# Autodesk Inventor assembly: a_frame_oko
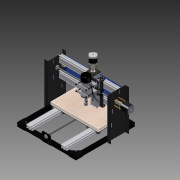
[picture p0: Inventor's stored thumbnail of the model, 180x180]
Saved by Autodesk Inventor 2014 (Build 180170000, 170)
## iProperties
Created: 2013-07-14
Part Number: a_frame_oko
Document SubType Name: Assembly
Designer: Edward
Mass: 4088.46 g
Surface Area: 15664.1 cm^2
Volume: 2491 cm^3
Density: 1.64129 g/cm^3
Author: Edward
## Documents named in this file (29)
- C:\Users\Edward\Desktop\Shapeoko_2.0_collection\Shapeoko_bm\a_frame_oko.iam
- C:\Users\Edward\Desktop\Shapeoko_2.0_collection\Shapeoko_bm\S2_MS400.ipt
- C:\Users\Edward\Desktop\Shapeoko_2.0_collection\Shapeoko_bm\hfs5_2020_400.ipt
- C:\Users\Edward\Desktop\Shapeoko_2.0_collection\Shapeoko_bm\x-carriage.ipt
- C:\Users\Edward\Desktop\Shapeoko_2.0_collection\Shapeoko_bm\y-carriage.ipt
- C:\Users\Edward\Desktop\Shapeoko_2.0_collection\Shapeoko_bm\hfs5_2020_360.ipt
- C:\Users\Edward\Desktop\Shapeoko_2.0_collection\Shapeoko_bm\SM-E01.ipt
- C:\Users\Edward\Desktop\Shapeoko_2.0_collection\Shapeoko_bm\SM-M08.ipt
- C:\Users\Edward\Desktop\Shapeoko_2.0_collection\Shapeoko_bm\B30037.iam
- C:\Users\Edward\Desktop\Shapeoko_2.0_collection\Shapeoko_bm\SM-H10.ipt
- C:\Users\Edward\Desktop\Shapeoko_2.0_collection\Shapeoko_bm\SM-H12.ipt
- C:\Users\Edward\Desktop\Shapeoko_2.0_collection\Shapeoko_bm\wasteboard.ipt
- C:\Users\Edward\Desktop\Shapeoko_2.0_collection\Shapeoko_bm\B18033.ipt
- C:\Users\Edward\Desktop\Shapeoko_2.0_collection\Shapeoko_bm\frame_gusset.ipt
- C:\Users\Edward\Desktop\Shapeoko_2.0_collection\Shapeoko_bm\93655A021.ipt
- C:\Users\Edward\Desktop\Shapeoko_2.0_collection\Shapeoko_bm\hblsd_assembly.iam
- C:\Users\Edward\Desktop\Shapeoko_2.0_collection\Shapeoko_bm\7804K145.ipt
- C:\Users\Edward\Desktop\Shapeoko_2.0_collection\Shapeoko_bm\part_plate_rear.ipt
- C:\Users\Edward\Desktop\Shapeoko_2.0_collection\Shapeoko_bm\91239A233.ipt
- C:\Users\Edward\Desktop\Shapeoko_2.0_collection\Shapeoko_bm\SM-H03.ipt
- C:\Users\Edward\Desktop\Shapeoko_2.0_collection\Shapeoko_bm\revamped_simple_z-axis_assembly.iam
- C:\Users\Edward\Desktop\Shapeoko_2.0_collection\Shapeoko_bm\simple_upright.ipt
- C:\Users\Edward\Desktop\Shapeoko_2.0_collection\Shapeoko_bm\z-bearing.ipt
- C:\Users\Edward\Desktop\Shapeoko_2.0_collection\Shapeoko_bm\nema17_y_axis_motor_mount_12ga.ipt
- C:\Users\Edward\Desktop\Shapeoko_2.0_collection\Shapeoko_bm\Imported Components\iec320_703W-00_04\iec320_703W-00_04.ipt
- C:\Users\Edward\Desktop\Shapeoko_2.0_collection\Shapeoko_bm\Imported Components\Arduino\Arduino.ipt
- C:\Users\Edward\Desktop\Shapeoko_2.0_collection\Shapeoko_bm\x_acme_upgrade.ipt
- C:\Users\Edward\Desktop\Shapeoko_2.0_collection\Shapeoko_bm\Imported Components\92844-005 USB CABLE B MALE TO B FEMALE PANEL MOUNT\92844-005 USB CABLE B MALE TO B FEMALE PANEL MOUNT.ipt
- C:\Users\Edward\Desktop\Shapeoko_2.0_collection\Shapeoko_bm\23015T81_leveling_feet.ipt
## Components (93 placed, 28 different names)
1. S2_MS400:1 — Mate:2, Flush:2, Flush:5, Mate:61, Flush:49, Mate:65, Flush:51
2. S2_MS400:2 — Mate:1, Flush:1, Mate:3, Flush:4, Mate:15, Mate:63, Flush:50, Mate:67, Flush:52
3. S2_MS400:3 — Flush:13, Flush:14, Flush:16, Angle:5, Insert:68, Insert:70
4. S2_MS400:4 — Flush:13, Flush:14, Mate:81, Flush:64, Mate:86, Flush:66, Insert:67, Flush:70, Insert:69, Mate:93, Flush:73
5. hfs5_2020_360:1 — Mate:1, Mate:2, Flush:1, Flush:2, Flush:3, Mate:4, Mate:5, Flush:6, Flush:7, Flush:8, Flush:9, Mate:39, Flush:33, Flush:37, Flush:40, Mate:64, Mate:66, Mate:95, Flush:74
6. hfs5_2020_360:2 — Mate:3, Flush:3, Flush:4, Flush:5, Flush:16, Mate:26, Flush:25, Flush:42, Flush:44, Flush:45, Flush:48, Mate:60, Mate:62
7. hfs5_2020_400:3 — Mate:4, Flush:8, Flush:9, Flush:34, Mate:45, Mate:54, Mate:55, Flush:46, Flush:47, Mate:90, Flush:71, Flush:77
8. hfs5_2020_400:4 — Mate:5, Flush:6, Flush:7, Flush:26, Mate:50, Mate:51, Flush:38, Flush:39, Mate:52, Flush:41, Mate:53, Flush:43, Mate:91, Flush:72
9. y-carriage:1 — Mate:15, Mate:20, Flush:20, Flush:21, Mate:36, Flush:31, Flush:32, Insert:3, Insert:4, Insert:5, Insert:6, Insert:7, Insert:8, Insert:9, Insert:10, Mate:41, Mate:44, Mate:57, Mate:59
10. SM-E01:2 — Mate:23, Insert:30, Insert:31, Insert:32, Insert:33, Mate:92, Mate:105
11. SM-M08:1 — Mate:20, Flush:20, Flush:21, Mate:28
12. SM-M08:2 — Mate:23, Flush:63, Mate:102
13. nema17_y_axis_motor_mount_12ga:1 — Mate:26, Flush:25, Flush:26, Angle:2, Mate:46, Angle:3, Angle:5, Insert:76, Flush:78
14. SM-E01:3 — Mate:28, Angle:2, Mate:30, Mate:46, Angle:3, Insert:20, Insert:21, Insert:24, Insert:25
15. SM-H12:1 — Mate:30, Mate:101
16. x_acme_upgrade:2 — Insert:81, Mate:101
17. x_acme_upgrade:1 — Mate:102, Insert:82
18. wasteboard:1 — Mate:36, Flush:31, Flush:32
19. B30037:5 [sub-assembly] — Insert:3
20. B30037:6 [sub-assembly] — Insert:4, Insert:64
21. B30037:7 [sub-assembly] — Insert:5, Insert:66
22. B30037:8 [sub-assembly] — Insert:6
23. B18033:1 — Insert:7, Mate:58
24. B18033:2 — Insert:8, Mate:56
25. B18033:3 — Insert:9, Mate:43
26. B18033:4 — Insert:10, Mate:40
27. B30037:9 [sub-assembly] — Mate:58, Mate:59, Insert:63
28. B30037:10 [sub-assembly] — Mate:40, Mate:41
29. B30037:11 [sub-assembly] — Mate:43, Mate:44
30. B30037:12 [sub-assembly] — Mate:56, Mate:57, Insert:65
31. frame_gusset:1 — Mate:39, Flush:33, Flush:34, Flush:35, Flush:36
32. frame_gusset:2 — Mate:45, Flush:35, Flush:36, Insert:83
33. frame_gusset:3 — Mate:51, Flush:37, Flush:38
34. frame_gusset:4 — Mate:50, Flush:39, Flush:40, Insert:84
35. frame_gusset:5 — Mate:52, Flush:41, Flush:42
36. frame_gusset:6 — Mate:53, Flush:43, Flush:44, Insert:85
37. frame_gusset:7 — Mate:55, Flush:45, Flush:46, Insert:86
38. frame_gusset:8 — Mate:54, Flush:47, Flush:48
39. 93655A021:1 — Insert:22
40. 93655A021:2 — Insert:19, Insert:21
41. 93655A021:3 — Insert:19
42. 93655A021:4 — Insert:18, Insert:20
43. 93655A021:5 — Insert:18
44. 93655A021:6 — Insert:22, Insert:25
45. 93655A021:7 — Insert:23
46. 93655A021:8 — Insert:23, Insert:24
47. hblsd_assembly:1 [sub-assembly] — Mate:64, Mate:65, Flush:51
48. hblsd_assembly:2 [sub-assembly] — Mate:66, Mate:67, Flush:52
49. hblsd_assembly:3 [sub-assembly] — Mate:62, Mate:63, Flush:50
50. hblsd_assembly:4 [sub-assembly] — Mate:60, Mate:61, Flush:49
51. 93655A021:9 — Insert:31
52. 93655A021:10
53. 93655A021:11 — Insert:33
54. 93655A021:12
55. 93655A021:13 — Insert:32
56. 93655A021:14
57. 93655A021:15 — Insert:30
58. 93655A021:16 — Insert:75
59. 7804K145:1 — Insert:55
60. B30037:14 [sub-assembly] — Insert:51
61. B30037:15 [sub-assembly] — Insert:52
62. x-carriage:2 — Mate:81, Flush:63, Flush:64, Insert:51, Insert:52, Insert:53, Insert:54, Mate:83, Mate:85, Mate:89, Flush:68, Flush:69
63. B18033:5 — Insert:53, Mate:84
64. B18033:6 — Insert:54, Mate:82
65. B30037:16 [sub-assembly] — Mate:82, Mate:83
66. B30037:17 [sub-assembly] — Mate:84, Mate:85
67. SM-H10:12 — Insert:55
68. part_plate_rear:1 — Mate:86, Flush:66
69. 91239A233:1 — Insert:59
70. SM-H03:1 — Insert:59, Insert:65
71. 91239A233:2
72. SM-H03:2 — Insert:63
73. 91239A233:3
74. SM-H03:3 — Insert:66
75. 91239A233:4
76. SM-H03:4 — Insert:64
77. revamped_simple_z-axis_assembly:1 [sub-assembly] — Mate:89, Flush:68, Flush:69
78. simple_upright:1 — Mate:90, Insert:67, Flush:70, Flush:71, Insert:68, Insert:71, Insert:75, Flush:77
79. simple_upright:2 — Mate:91, Flush:72, Insert:69, Insert:70, Insert:72, Mate:97, Flush:76, Mate:98, Mate:103
80. z-bearing:1 — Insert:71
81. z-bearing:2 — Insert:72, Mate:92, Insert:82
82. part_plate_rear:2 — Mate:93, Flush:73, Mate:100, Flush:79
83. z-bearing:3 — Insert:76
84. nema17_y_axis_motor_mount_12ga:2 — Insert:78, Mate:95, Flush:74, Flush:78
85. z-bearing:4 — Insert:78, Insert:81
86. SM-H12:3 — Mate:105
87. iec320_703W-00_04:1 — Mate:97, Flush:76, Mate:98
88. Arduino:1 — Mate:100, Flush:79
89. 92844-005 USB CABLE B MALE TO B FEMALE PANEL MOUNT:1 — Mate:103
90. 23015T81_leveling_feet:1 — Insert:83
91. 23015T81_leveling_feet:2 — Insert:84
92. 23015T81_leveling_feet:3 — Insert:85
93. 23015T81_leveling_feet:4 — Insert:86
## Relationships (163: Mate 56, Flush 52, Insert 52, Angle 3)
- Mate:1: S2_MS400:2 ↔ hfs5_2020_360:1
- Mate:2: S2_MS400:1 ↔ hfs5_2020_360:1
- Flush:1: S2_MS400:2 ↔ hfs5_2020_360:1
- Flush:2: S2_MS400:1 ↔ hfs5_2020_360:1
- Mate:3: S2_MS400:2 ↔ hfs5_2020_360:2
- Flush:3: hfs5_2020_360:1 ↔ hfs5_2020_360:2
- Flush:4: S2_MS400:2 ↔ hfs5_2020_360:2
- Flush:5: S2_MS400:1 ↔ hfs5_2020_360:2
- Mate:4: hfs5_2020_360:1 ↔ hfs5_2020_400:3
- Mate:5: hfs5_2020_360:1 ↔ hfs5_2020_400:4
- Flush:6: hfs5_2020_360:1 ↔ hfs5_2020_400:4
- Flush:7: hfs5_2020_360:1 ↔ hfs5_2020_400:4
- Flush:8: hfs5_2020_360:1 ↔ hfs5_2020_400:3
- Flush:9: hfs5_2020_360:1 ↔ hfs5_2020_400:3
- Flush:13: S2_MS400:3 ↔ S2_MS400:4
- Flush:14 (90 mm): S2_MS400:3 ↔ S2_MS400:4
- Mate:15 (6.35 mm): S2_MS400:2 ↔ y-carriage:1
- Flush:16 (95.5 mm): S2_MS400:3 ↔ hfs5_2020_360:2
- Mate:20: y-carriage:1 ↔ SM-M08:1
- Flush:20 (90 mm): y-carriage:1 ↔ SM-M08:1
- Flush:21 (142.5 mm): y-carriage:1 ↔ SM-M08:1
- Mate:23: SM-E01:2 ↔ SM-M08:2
- Mate:26: hfs5_2020_360:2 ↔ nema17_y_axis_motor_mount_12ga:1
- Flush:25: hfs5_2020_360:2 ↔ nema17_y_axis_motor_mount_12ga:1
- Flush:26 (170 mm): hfs5_2020_400:4 ↔ nema17_y_axis_motor_mount_12ga:1
- Mate:28: SM-M08:1 ↔ SM-E01:3
- Angle:2 (0 deg): nema17_y_axis_motor_mount_12ga:1 ↔ SM-E01:3
- Mate:30: SM-E01:3 ↔ SM-H12:1
- Mate:36: y-carriage:1 ↔ wasteboard:1
- Flush:31: y-carriage:1 ↔ wasteboard:1
- Flush:32: y-carriage:1 ↔ wasteboard:1
- Insert:3 (1 mm): y-carriage:1 ↔ B30037:5
- Insert:4 (1 mm): y-carriage:1 ↔ B30037:6
- Insert:5 (1 mm): y-carriage:1 ↔ B30037:7
- Insert:6 (1 mm): y-carriage:1 ↔ B30037:8
- Insert:7: y-carriage:1 ↔ B18033:1
- Insert:8: y-carriage:1 ↔ B18033:2
- Insert:9: y-carriage:1 ↔ B18033:3
- Insert:10: y-carriage:1 ↔ B18033:4
- Mate:39: hfs5_2020_360:1 ↔ frame_gusset:1
- Flush:33: hfs5_2020_360:1 ↔ frame_gusset:1
- Flush:34: hfs5_2020_400:3 ↔ frame_gusset:1
- Mate:40: B18033:4 ↔ B30037:10
- Mate:41 (1 mm): y-carriage:1 ↔ B30037:10
- Mate:43: B18033:3 ↔ B30037:11
- Mate:44 (1 mm): y-carriage:1 ↔ B30037:11
- Mate:45: hfs5_2020_400:3 ↔ frame_gusset:2
- Flush:35: frame_gusset:1 ↔ frame_gusset:2
- Flush:36: frame_gusset:1 ↔ frame_gusset:2
- Mate:46 (50 mm): nema17_y_axis_motor_mount_12ga:1 ↔ SM-E01:3
- Angle:3 (0 deg): nema17_y_axis_motor_mount_12ga:1 ↔ SM-E01:3
- Mate:50: hfs5_2020_400:4 ↔ frame_gusset:4
- Mate:51: hfs5_2020_400:4 ↔ frame_gusset:3
- Flush:37: hfs5_2020_360:1 ↔ frame_gusset:3
- Flush:38: hfs5_2020_400:4 ↔ frame_gusset:3
- Flush:39: hfs5_2020_400:4 ↔ frame_gusset:4
- Flush:40: hfs5_2020_360:1 ↔ frame_gusset:4
- Mate:52: hfs5_2020_400:4 ↔ frame_gusset:5
- Flush:41: hfs5_2020_400:4 ↔ frame_gusset:5
- Flush:42: hfs5_2020_360:2 ↔ frame_gusset:5
- Mate:53: hfs5_2020_400:4 ↔ frame_gusset:6
- Flush:43: hfs5_2020_400:4 ↔ frame_gusset:6
- Flush:44: hfs5_2020_360:2 ↔ frame_gusset:6
- Mate:54: hfs5_2020_400:3 ↔ frame_gusset:8
- Mate:55: hfs5_2020_400:3 ↔ frame_gusset:7
- Flush:45: hfs5_2020_360:2 ↔ frame_gusset:7
- Flush:46: hfs5_2020_400:3 ↔ frame_gusset:7
- Flush:47: hfs5_2020_400:3 ↔ frame_gusset:8
- Flush:48: hfs5_2020_360:2 ↔ frame_gusset:8
- Mate:56: B18033:2 ↔ B30037:12
- Mate:57 (1 mm): y-carriage:1 ↔ B30037:12
- Mate:58: B18033:1 ↔ B30037:9
- Mate:59 (1 mm): y-carriage:1 ↔ B30037:9
- Insert:18: 93655A021:4 ↔ 93655A021:5
- Insert:19: 93655A021:2 ↔ 93655A021:3
- Insert:20: SM-E01:3 ↔ 93655A021:4
- Insert:21: SM-E01:3 ↔ 93655A021:2
- Insert:22: 93655A021:1 ↔ 93655A021:6
- Insert:23: 93655A021:7 ↔ 93655A021:8
- Insert:24: SM-E01:3 ↔ 93655A021:8
- Insert:25: SM-E01:3 ↔ 93655A021:6
- Mate:60: hfs5_2020_360:2 ↔ hblsd_assembly:4
- Mate:61: S2_MS400:1 ↔ hblsd_assembly:4
- Flush:49 (3 mm): S2_MS400:1 ↔ hblsd_assembly:4
- Mate:62: hfs5_2020_360:2 ↔ hblsd_assembly:3
- Mate:63: S2_MS400:2 ↔ hblsd_assembly:3
- Flush:50 (3 mm): S2_MS400:2 ↔ hblsd_assembly:3
- Mate:64: hfs5_2020_360:1 ↔ hblsd_assembly:1
- Mate:65: S2_MS400:1 ↔ hblsd_assembly:1
- Flush:51 (3 mm): S2_MS400:1 ↔ hblsd_assembly:1
- Mate:66: hfs5_2020_360:1 ↔ hblsd_assembly:2
- Mate:67: S2_MS400:2 ↔ hblsd_assembly:2
- Flush:52 (3 mm): S2_MS400:2 ↔ hblsd_assembly:2
- [Insert]: 93655A021:9 ↔ 93655A021:10
- [Insert]: 93655A021:11 ↔ 93655A021:12
- [Insert]: 93655A021:13 ↔ 93655A021:14
- [Insert]: 93655A021:15 ↔ 93655A021:16
- Insert:30: SM-E01:2 ↔ 93655A021:15
- Insert:31: SM-E01:2 ↔ 93655A021:9
- Insert:32: SM-E01:2 ↔ 93655A021:13
- Insert:33: SM-E01:2 ↔ 93655A021:11
- Angle:5 (0 deg): S2_MS400:3 ↔ nema17_y_axis_motor_mount_12ga:1
- Mate:81 (6.35 mm): S2_MS400:4 ↔ x-carriage:2
- Flush:63: SM-M08:2 ↔ x-carriage:2
- Flush:64 (-22.5 mm): S2_MS400:4 ↔ x-carriage:2
- Insert:51 (1 mm): B30037:14 ↔ x-carriage:2
- Insert:52 (1 mm): B30037:15 ↔ x-carriage:2
- Insert:53: x-carriage:2 ↔ B18033:5
- Insert:54: x-carriage:2 ↔ B18033:6
- Mate:82: B18033:6 ↔ B30037:16
- Mate:83 (1 mm): x-carriage:2 ↔ B30037:16
- Mate:84: B18033:5 ↔ B30037:17
- Mate:85 (1 mm): x-carriage:2 ↔ B30037:17
- Insert:55: 7804K145:1 ↔ SM-H10:12
- Mate:86 (6.35 mm): S2_MS400:4 ↔ part_plate_rear:1
- Flush:66: S2_MS400:4 ↔ part_plate_rear:1
- Insert:59: 91239A233:1 ↔ SM-H03:1
- [Insert]: 91239A233:2 ↔ SM-H03:2
- [Insert]: 91239A233:3 ↔ SM-H03:3
- [Insert]: 91239A233:4 ↔ SM-H03:4
- Insert:63: B30037:9 ↔ SM-H03:2
- Insert:64: B30037:6 ↔ SM-H03:4
- Insert:65: B30037:12 ↔ SM-H03:1
- Insert:66: B30037:7 ↔ SM-H03:3
- Mate:89: x-carriage:2 ↔ revamped_simple_z-axis_assembly:1
- Flush:68 (20 mm): x-carriage:2 ↔ revamped_simple_z-axis_assembly:1
- Flush:69: x-carriage:2 ↔ revamped_simple_z-axis_assembly:1
- Mate:90: hfs5_2020_400:3 ↔ simple_upright:1
- Insert:67: S2_MS400:4 ↔ simple_upright:1
- Flush:70: S2_MS400:4 ↔ simple_upright:1
- Flush:71: hfs5_2020_400:3 ↔ simple_upright:1
- Insert:68: S2_MS400:3 ↔ simple_upright:1
- Mate:91: hfs5_2020_400:4 ↔ simple_upright:2
- Flush:72: hfs5_2020_400:4 ↔ simple_upright:2
- Insert:69: S2_MS400:4 ↔ simple_upright:2
- Insert:70: S2_MS400:3 ↔ simple_upright:2
- Insert:71: simple_upright:1 ↔ z-bearing:1
- Insert:72: simple_upright:2 ↔ z-bearing:2
- Mate:92: SM-E01:2 ↔ z-bearing:2
- Insert:75: 93655A021:16 ↔ simple_upright:1
- Mate:93: S2_MS400:4 ↔ part_plate_rear:2
- Flush:73: S2_MS400:4 ↔ part_plate_rear:2
- Insert:76: nema17_y_axis_motor_mount_12ga:1 ↔ z-bearing:3
- Insert:78: nema17_y_axis_motor_mount_12ga:2 ↔ z-bearing:4
- Mate:95: hfs5_2020_360:1 ↔ nema17_y_axis_motor_mount_12ga:2
- Flush:74: hfs5_2020_360:1 ↔ nema17_y_axis_motor_mount_12ga:2
- Mate:97: simple_upright:2 ↔ iec320_703W-00_04:1
- Flush:76 (50 mm): simple_upright:2 ↔ iec320_703W-00_04:1
- Mate:98 (10 mm): simple_upright:2 ↔ iec320_703W-00_04:1
- Flush:77: hfs5_2020_400:3 ↔ simple_upright:1
- Flush:78: nema17_y_axis_motor_mount_12ga:1 ↔ nema17_y_axis_motor_mount_12ga:2
- Mate:100: part_plate_rear:2 ↔ Arduino:1
- Flush:79 (35 mm): part_plate_rear:2 ↔ Arduino:1
- Insert:81: x_acme_upgrade:2 ↔ z-bearing:4
- Mate:101: SM-H12:1 ↔ x_acme_upgrade:2
- Mate:102: SM-M08:2 ↔ x_acme_upgrade:1
- Insert:82: x_acme_upgrade:1 ↔ z-bearing:2
- Mate:103: simple_upright:2 ↔ 92844-005 USB CABLE B MALE TO B FEMALE PANEL MOUNT:1
- Insert:83 (4 mm): frame_gusset:2 ↔ 23015T81_leveling_feet:1
- Insert:84 (4 mm): frame_gusset:4 ↔ 23015T81_leveling_feet:2
- Insert:85 (4 mm): frame_gusset:6 ↔ 23015T81_leveling_feet:3
- Insert:86 (4 mm): frame_gusset:7 ↔ 23015T81_leveling_feet:4
- Mate:105: SM-E01:2 ↔ SM-H12:3
## Named parameters: d148_d129 = 0 mm, d149_d129 = 0 mm, d150_d129 = 0 mm, d151_d129 = 0 mm, d229_d228 = 0 mm, d230_d228 = 0 mm, d231_d228 = 0 mm, d269_d266 = 0 mm
